# Autodesk Inventor assembly: Assembly146-01
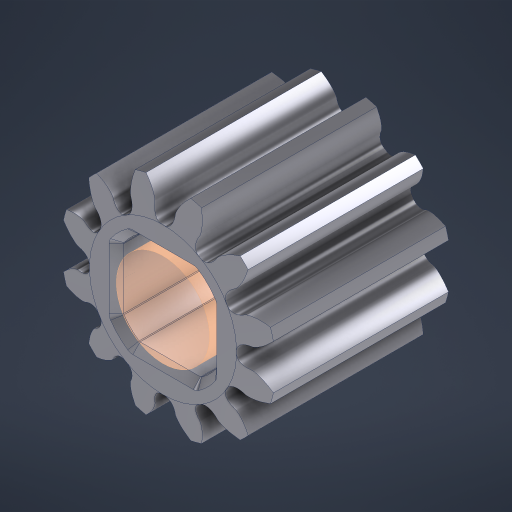
[picture p0: Inventor's stored thumbnail of the model, 512x512]
Saved by Autodesk Inventor 2024 (Build 280153000, 153)
## iProperties
Created: 2022-08-02
Part Number: Assembly146-01
Document SubType Name: Assembly
Designer: ylu12
Author: ylu12
## Documents named in this file (3)
- C:\Users\avere\Documents\rbp_cad\VEX-CAD-Inventor-1.41\Motion\Gears\HS Gear\HS 12T Gear, No Insert.iam
- C:\Users\avere\Documents\rbp_cad\VEX-CAD-Inventor-1.41\Motion\Gears\Reference Files\HS 12T Gear, No Insert.ipt
- C:\Users\avere\Documents\rbp_cad\VEX-CAD-Inventor-1.41\Motion\Gears\HS Gear.iam
## Components (1 placed, 1 different names)
1. 12T — Mate:5, Mate:6, Flush:3
## Relationships (3: Mate 2, Flush 1)
- Mate:5: 12T
- Mate:6: 12T
- Flush:3: 12T
